# Autodesk Inventor assembly: Bearing Assembly (both end holes)
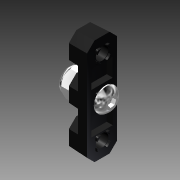
[picture p0: Inventor's stored thumbnail of the model, 180x180]
Saved by Autodesk Inventor 2012 (Build 160160000, 160)
## iProperties
Created: 2011-09-10
Part Number: Bearing Assembly (both end holes)
Document SubType Name: Assembly
Designer: Wade
Author: Wade
## Documents named in this file (4)
- C:\Users\Wade\Documents\1103 Robot - CAD Assembly\Bearing Assembly (both end holes).iam
- C:\Users\Wade\Documents\24C VEX CAD Files\Other Parts\Bearing Flat, Delrin.ipt
- C:\Users\Wade\Documents\24C VEX CAD Files\Screws & Nuts\Screw 8-32 x 0.500''-Silver.ipt
- C:\Users\Wade\Documents\24C VEX CAD Files\Screws & Nuts\Nut 8-32 Nylock.ipt
## Components (3 placed, 3 different names)
1. Bearing Flat, Delrin:1 — Mate:2, Mate:4, Mate:8
2. Screw 8-32 x 0.500''-Silver:2 — Mate:2, Mate:4, Mate:6
3. Nut 8-32 Nylock:2 — Mate:6, Mate:8
## Relationships (4: Mate 4)
- Mate:2: Bearing Flat, Delrin:1 ↔ Screw 8-32 x 0.500''-Silver:2
- Mate:4 (1.1684 mm): Bearing Flat, Delrin:1 ↔ Screw 8-32 x 0.500''-Silver:2
- Mate:6: Screw 8-32 x 0.500''-Silver:2 ↔ Nut 8-32 Nylock:2
- Mate:8: Bearing Flat, Delrin:1 ↔ Nut 8-32 Nylock:2
